# Autodesk Inventor assembly: Germination
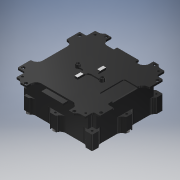
[picture p0: Inventor's stored thumbnail of the model, 180x180]
Saved by Autodesk Inventor 2018 (Build 220112000, 112)
## iProperties
Created: 2020-10-06
Part Number: Germination
Document SubType Name: Assembly
Designer: Bradley
Author: Bradley
## Documents named in this file (5)
- C:\Users\Bradley\Documents\GitHub\CougSat1-Hardware\CougSat1-Payload\CADModel\Imported\Germination.iam
- C:\Users\Bradley\Documents\GitHub\CougSat1-Hardware\CougSat1-Payload\CADModel\Imported\Germination_Bottom.ipt
- C:\Users\Bradley\Documents\GitHub\CougSat1-Hardware\CougSat1-Payload\CADModel\Imported\Germination_Top.ipt
- C:\Users\Bradley\Documents\GitHub\Resources\SupplierDocuments\48 - Hardware\48-0362\48-0362.ipt
- C:\Users\Bradley\Documents\GitHub\Resources\SupplierDocuments\48 - Hardware\48-0361\48-0361.ipt
## Components (11 placed, 4 different names)
1. Germination_Bottom:1 — Insert:1, Insert:2, Insert:3, Insert:4, Insert:5, Insert:6, Insert:7, Insert:8, Insert:9, Insert:10, Insert:11
2. Germination_Top:1 — Insert:9, Insert:10
3. 48-0362:1 — Insert:1
4. 48-0361:1 — Insert:2
5. 48-0361:2 — Insert:4
6. 48-0362:2 — Insert:5
7. 48-0361:3 — Insert:8
8. 48-0362:3 — Insert:6
9. 48-0361:4 — Insert:7
10. 48-0361:5 — Insert:3
11. 48-0361:6 — Insert:11
## Relationships (11: Insert 11)
- Insert:1: Germination_Bottom:1 ↔ 48-0362:1
- Insert:2: Germination_Bottom:1 ↔ 48-0361:1
- Insert:3: Germination_Bottom:1 ↔ 48-0361:5
- Insert:4: Germination_Bottom:1 ↔ 48-0361:2
- Insert:5: Germination_Bottom:1 ↔ 48-0362:2
- Insert:6: Germination_Bottom:1 ↔ 48-0362:3
- Insert:7: Germination_Bottom:1 ↔ 48-0361:4
- Insert:8: Germination_Bottom:1 ↔ 48-0361:3
- Insert:9: Germination_Bottom:1 ↔ Germination_Top:1
- Insert:10: Germination_Bottom:1 ↔ Germination_Top:1
- Insert:11: Germination_Bottom:1 ↔ 48-0361:6
